# Autodesk Inventor assembly: GFRP_T2_06
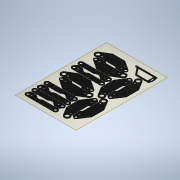
[picture p0: Inventor's stored thumbnail of the model, 180x180]
Saved by Autodesk Inventor 2020 (Build 240168000, 168)
## iProperties
Created: 2021-08-27
Part Number: GFRP_T2_06
Document SubType Name: Assembly
Designer: Masato
Author: Masato
## Documents named in this file (5)
- C:\Users\naoki\Documents\Inventor\CitBrains\git_clone\SUSTAINA_ver1_0\A_T2_175\SUSTAINA-OP\Cam\GFRP_T2_06.iam
- C:\Users\naoki\Documents\Inventor\CitBrains\git_clone\SUSTAINA_ver1_0\A_T2_175\SUSTAINA-OP\Cam\DisposableBoard.ipt
- C:\Users\naoki\Documents\Inventor\CitBrains\git_clone\SUSTAINA_ver1_0\A_T2_175\SUSTAINA-OP\LowerBody\Link\BackLink_frame.ipt
- C:\Users\naoki\Documents\Inventor\CitBrains\git_clone\SUSTAINA_ver1_0\A_T2_175\SUSTAINA-OP\LowerBody\Link\FrontLink_frame.ipt
- C:\Users\naoki\Documents\Inventor\CitBrains\git_clone\SUSTAINA_ver1_0\A_T2_175\SUSTAINA-OP\UpperBody\Arm\UpperArm_side_frame.ipt
## Components (16 placed, 4 different names)
1. DisposableBoard:1 — メイト:2, メイト:1, フラッシュ:1, フラッシュ:2, メイト:4, メイト:5, 正接:1, 正接:2, メイト:9, 正接:5, メイト:15, 角度:1, メイト:18, メイト:19, 角度:2, 角度:3, 角度:4, メイト:25, メイト:26, フラッシュ:3, メイト:28, 正接:8, メイト:29, 正接:9, メイト:31, フラッシュ:4, 正接:16
2. FrontLink_frame:2 — メイト:9, 正接:5, 正接:7, メイト:17, 正接:17
3. FrontLink_frame:6 — メイト:16, メイト:18, 正接:10, 正接:12, 正接:13
4. UpperArm_side_frame:1 — メイト:15, 角度:1, 正接:14, フラッシュ:4
5. FrontLink_frame:7 — メイト:16, メイト:19, 角度:4, 正接:13, 正接:14
6. FrontLink_frame:8 — メイト:17, 角度:3, メイト:31, 正接:12, 正接:17
7. BackLink_frame:5 — メイト:27, フラッシュ:3, メイト:28, 正接:8
8. BackLink_frame:6 — メイト:27, メイト:29, 正接:9, メイト:30
9. FrontLink_frame:10 — メイト:23, メイト:26, 正接:15, 正接:16
10. FrontLink_frame:9 — メイト:20, メイト:23, メイト:25, 正接:15
11. BackLink_frame:1 — メイト:4, メイト:6, 正接:2, 正接:7, メイト:20
12. BackLink_frame:2 — メイト:5, メイト:6, 正接:1, 角度:2, メイト:30
13. FrontLink_frame:11
14. FrontLink_frame:12
15. BackLink_frame:3
16. BackLink_frame:4 — 正接:10
## Component patterns: (2 elements, first: FrontLink_frame:10 + FrontLink_frame:9 + BackLink_frame:1 + BackLink_frame:2)
## Relationships (41: Mate 20, Tangent 13, Flush 4, Angle 4)
- メイト:2 [Mate]: DisposableBoard:1
- メイト:1 [Mate]: DisposableBoard:1
- フラッシュ:1 [Flush]: DisposableBoard:1
- フラッシュ:2 [Flush]: DisposableBoard:1
- メイト:4 [Mate]: DisposableBoard:1 ↔ BackLink_frame:1
- メイト:5 [Mate]: DisposableBoard:1 ↔ BackLink_frame:2
- メイト:6 [Mate] (2.5 mm): BackLink_frame:1 ↔ BackLink_frame:2
- 正接:1 [Tangent] (2 mm): DisposableBoard:1 ↔ BackLink_frame:2
- 正接:2 [Tangent] (2 mm): DisposableBoard:1 ↔ BackLink_frame:1
- メイト:9 [Mate]: DisposableBoard:1 ↔ FrontLink_frame:2
- 正接:5 [Tangent] (2.5 mm): DisposableBoard:1 ↔ FrontLink_frame:2
- 正接:7 [Tangent] (2.5 mm): FrontLink_frame:2 ↔ BackLink_frame:1
- メイト:15 [Mate]: DisposableBoard:1 ↔ UpperArm_side_frame:1
- 角度:1 [Angle] (0 deg): DisposableBoard:1 ↔ UpperArm_side_frame:1
- メイト:16 [Mate] (2.5 mm): FrontLink_frame:6 ↔ FrontLink_frame:7
- メイト:17 [Mate] (2.5 mm): FrontLink_frame:2 ↔ FrontLink_frame:8
- メイト:18 [Mate]: DisposableBoard:1 ↔ FrontLink_frame:6
- メイト:19 [Mate]: DisposableBoard:1 ↔ FrontLink_frame:7
- 角度:2 [Angle] (0 deg): DisposableBoard:1 ↔ BackLink_frame:2
- 角度:3 [Angle] (0 deg): DisposableBoard:1 ↔ FrontLink_frame:8
- 角度:4 [Angle] (0 deg): DisposableBoard:1 ↔ FrontLink_frame:7
- メイト:20 [Mate] (2.5 mm): FrontLink_frame:9 ↔ BackLink_frame:1
- メイト:23 [Mate] (2.5 mm): FrontLink_frame:10 ↔ FrontLink_frame:9
- メイト:25 [Mate]: DisposableBoard:1 ↔ FrontLink_frame:9
- メイト:26 [Mate]: DisposableBoard:1 ↔ FrontLink_frame:10
- メイト:27 [Mate] (2.5 mm): BackLink_frame:5 ↔ BackLink_frame:6
- フラッシュ:3 [Flush] (2 mm): DisposableBoard:1 ↔ BackLink_frame:5
- メイト:28 [Mate]: DisposableBoard:1 ↔ BackLink_frame:5
- 正接:8 [Tangent] (2 mm): DisposableBoard:1 ↔ BackLink_frame:5
- メイト:29 [Mate]: DisposableBoard:1 ↔ BackLink_frame:6
- 正接:9 [Tangent] (2 mm): DisposableBoard:1 ↔ BackLink_frame:6
- メイト:30 [Mate] (2.5 mm): BackLink_frame:6 ↔ BackLink_frame:2
- 正接:10 [Tangent] (2.5 mm): FrontLink_frame:6 ↔ BackLink_frame:4
- メイト:31 [Mate]: DisposableBoard:1 ↔ FrontLink_frame:8
- 正接:12 [Tangent] (2.5 mm): FrontLink_frame:6 ↔ FrontLink_frame:8
- 正接:13 [Tangent] (3 mm): FrontLink_frame:6 ↔ FrontLink_frame:7
- 正接:14 [Tangent] (2.5 mm): UpperArm_side_frame:1 ↔ FrontLink_frame:7
- フラッシュ:4 [Flush] (4 mm): DisposableBoard:1 ↔ UpperArm_side_frame:1
- 正接:15 [Tangent] (3 mm): FrontLink_frame:10 ↔ FrontLink_frame:9
- 正接:16 [Tangent] (2 mm): DisposableBoard:1 ↔ FrontLink_frame:10
- 正接:17 [Tangent] (3 mm): FrontLink_frame:2 ↔ FrontLink_frame:8
